# Autodesk Inventor assembly: Manfrotto Logo 01
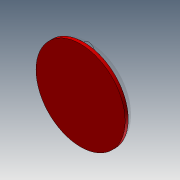
[picture p0: Inventor's stored thumbnail of the model, 180x180]
Saved by Autodesk Inventor 2011 (Build 150239000, 239)
## iProperties
Created: 2012-11-06
Part Number: Manfrotto Logo 01
Document SubType Name: Assembly
Designer: Lance
Author: Lance
## Documents named in this file (3)
- C:\Inventor Projects\MPX0032 - Projector Accessories\Manfrotto 494RC2 - Tripod Head\Manfrotto Logo 01.iam
- C:\Inventor Projects\MPX0032 - Projector Accessories\Manfrotto 494RC2 - Tripod Head\Manfrotto Logo 01 - 1.ipt
- C:\Inventor Projects\MPX0032 - Projector Accessories\Manfrotto 494RC2 - Tripod Head\Manfrotto Logo 01 - 2.ipt
## Components (2 placed, 2 different names)
1. Manfrotto Logo 01 - 1:1 — Insert:1, Angle:1
2. Manfrotto Logo 01 - 2:1 — Insert:1, Angle:1
## Relationships (2: Insert 1, Angle 1)
- Insert:1: Manfrotto Logo 01 - 1:1 ↔ Manfrotto Logo 01 - 2:1
- Angle:1 (180 deg): Manfrotto Logo 01 - 1:1 ↔ Manfrotto Logo 01 - 2:1
